# Autodesk Inventor assembly: 4K shield
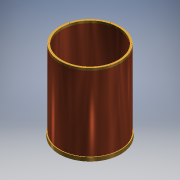
[picture p0: Inventor's stored thumbnail of the model, 180x180]
Saved by Autodesk Inventor 2018 (Build 220112000, 112)
## iProperties
Created: 2019-03-06
Part Number: 4K shield
Document SubType Name: Assembly
Designer: Admin
Author: Admin
## Documents named in this file (4)
- C:\Users\Admin\Documents\Cryostat\CAD\4K shield.iam
- C:\Users\Admin\Documents\Cryostat\CAD\4K sheild rim.ipt
- C:\Users\Admin\Documents\Cryostat\CAD\4K sheild body.ipt
- C:\Users\Admin\Documents\Cryostat\CAD\4K sheild rim2.ipt
## Components (3 placed, 3 different names)
1. 4K sheild rim:1 — Mate:1, Mate:2
2. 4K sheild body:1 — Mate:1, Mate:2, Mate:3, Mate:4
3. 4K sheild rim2:1 — Mate:3, Mate:4
## Relationships (4: Mate 4)
- Mate:1: 4K sheild rim:1 ↔ 4K sheild body:1
- Mate:2: 4K sheild rim:1 ↔ 4K sheild body:1
- Mate:3: 4K sheild body:1 ↔ 4K sheild rim2:1
- Mate:4: 4K sheild body:1 ↔ 4K sheild rim2:1
